# Autodesk Inventor assembly: Manipulator Bent Shields
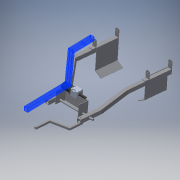
[picture p0: Inventor's stored thumbnail of the model, 180x180]
Saved by Autodesk Inventor 2017 (Build 210142000, 142)
## iProperties
Created: 2019-02-04
Part Number: Manipulator Bent Shields
Document SubType Name: Assembly
Designer: S346553810
Author: S346553810
## Documents named in this file (10)
- \\ad.ocdsb.ca\studenthome\5\S346795925\frc-season-2019-deep-space-1\Robot\Robot\Manipulator Bent Shields.iam
- \\ad.ocdsb.ca\studenthome\5\S346795925\frc-season-2019-deep-space-1\Robot\Robot\flap.ipt
- \\ad.ocdsb.ca\studenthome\5\S346795925\frc-season-2019-deep-space-1\Robot\Robot\Arm 2.ipt
- \\ad.ocdsb.ca\studenthome\5\S346795925\frc-season-2019-deep-space-1\Robot\Robot\Arm 2_MIR.ipt
- \\ad.ocdsb.ca\studenthome\5\S346795925\frc-season-2019-deep-space-1\Robot\Robot\Arm Hatch.ipt
- \\ad.ocdsb.ca\studenthome\5\S346795925\frc-season-2019-deep-space-1\Robot\Robot\VersaPlanetary_v1_Single_Stage_10_1_with_BAG.ipt
- \\ad.ocdsb.ca\studenthome\5\S346795925\frc-season-2019-deep-space-1\Robot\Robot\C chanel Short.ipt
- \\ad.ocdsb.ca\studenthome\5\S346795925\frc-season-2019-deep-space-1\Robot\Robot\Spinning Rod.ipt
- \\ad.ocdsb.ca\studenthome\5\S346795925\frc-season-2019-deep-space-1\Robot\Robot\Roller holder.ipt
- \\ad.ocdsb.ca\studenthome\5\S346795925\frc-season-2019-deep-space-1\Robot\Robot\Roller holder_CPY.ipt
## Components (12 placed, 9 different names)
1. flap:3 — Mate:6, Flush:1, Mate:33
2. flap:4 — Mate:5, Flush:2, Mate:7
3. Arm 2:2 — Mate:5, Flush:2, Mate:7, Mate:8, Flush:4, Mate:20, Mate:26, Flush:7, Mate:34, Flush:9, Flush:10, Mate:36, Flush:13, Mate:37
4. Arm 2_MIR:1 — Mate:6, Flush:1, Mate:8, Flush:4, Mate:18, Mate:27, Mate:32, Mate:33, Mate:35, Flush:11, Flush:12, Mate:38, Flush:14, Mate:39
5. Arm Hatch:1 — Mate:18, Mate:20
6. VersaPlanetary_v1_Single_Stage_10_1_with_BAG:1 — Mate:29, Mate:30, Flush:8
7. C chanel Short:1 — Mate:26, Mate:27, Mate:29, Mate:31, Mate:30, Flush:8, Mate:32
8. Spinning Rod:1 — Mate:31, Flush:7
9. Roller holder:1 — Mate:34, Flush:9, Flush:10
10. Roller holder:2 — Mate:35, Flush:11, Flush:12
11. Roller holder_CPY:1 — Mate:38, Flush:14, Mate:39
12. Roller holder_CPY:2 — Mate:36, Flush:13, Mate:37
## Relationships (30: Mate 19, Flush 11)
- Mate:5: flap:4 ↔ Arm 2:2
- Mate:6: flap:3 ↔ Arm 2_MIR:1
- Flush:1: flap:3 ↔ Arm 2_MIR:1
- Flush:2: flap:4 ↔ Arm 2:2
- Mate:7: flap:4 ↔ Arm 2:2
- Mate:8 (202.565 mm): Arm 2:2 ↔ Arm 2_MIR:1
- Flush:4: Arm 2:2 ↔ Arm 2_MIR:1
- Mate:18: Arm 2_MIR:1 ↔ Arm Hatch:1
- Mate:20: Arm 2:2 ↔ Arm Hatch:1
- Mate:26: Arm 2:2 ↔ C chanel Short:1
- Mate:27: Arm 2_MIR:1 ↔ C chanel Short:1
- Mate:29: VersaPlanetary_v1_Single_Stage_10_1_with_BAG:1 ↔ C chanel Short:1
- Mate:30 (-120.65 mm): VersaPlanetary_v1_Single_Stage_10_1_with_BAG:1 ↔ C chanel Short:1
- Mate:31: C chanel Short:1 ↔ Spinning Rod:1
- Flush:7 (-25.4 mm): Arm 2:2 ↔ Spinning Rod:1
- Flush:8: VersaPlanetary_v1_Single_Stage_10_1_with_BAG:1 ↔ C chanel Short:1
- Mate:32 (13.97 mm): Arm 2_MIR:1 ↔ C chanel Short:1
- Mate:33: flap:3 ↔ Arm 2_MIR:1
- Mate:34: Arm 2:2 ↔ Roller holder:1
- Flush:9: Arm 2:2 ↔ Roller holder:1
- Flush:10 (152.4 mm): Arm 2:2 ↔ Roller holder:1
- Mate:35: Arm 2_MIR:1 ↔ Roller holder:2
- Flush:11: Arm 2_MIR:1 ↔ Roller holder:2
- Flush:12 (152.4 mm): Arm 2_MIR:1 ↔ Roller holder:2
- Mate:36: Arm 2:2 ↔ Roller holder_CPY:2
- Flush:13: Arm 2:2 ↔ Roller holder_CPY:2
- Mate:37: Arm 2:2 ↔ Roller holder_CPY:2
- Mate:38: Arm 2_MIR:1 ↔ Roller holder_CPY:1
- Flush:14: Arm 2_MIR:1 ↔ Roller holder_CPY:1
- Mate:39: Arm 2_MIR:1 ↔ Roller holder_CPY:1
